# Autodesk Inventor assembly: Scrambler II
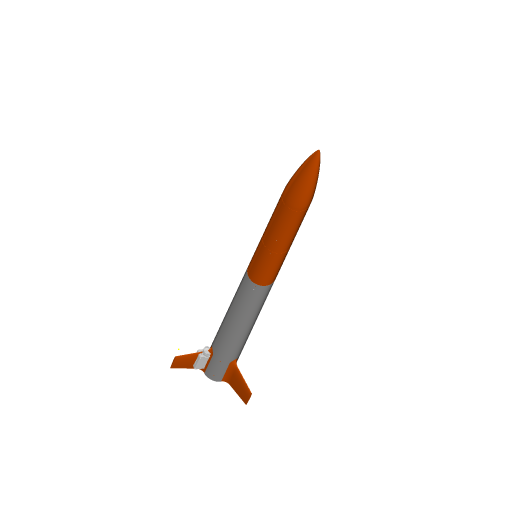
[picture p0: Inventor's stored thumbnail of the model, 512x512]
Saved by Autodesk Inventor 2024 (Build 280153000, 153)
## iProperties
Created: 2023-12-30
Part Number: Scrambler II
Document SubType Name: Assembly
Designer: Jamie
Mass: 631.455 g
Surface Area: 5625.65 cm^2
Volume: 391.502 cm^3
Density: 1.6129 g/cm^3
Author: Jamie
## Documents named in this file (7)
- C:\Users\Jamie\Documents\Uni\DARE\Scrambler-2-CAD\Autodesk\Scrambler II.iam
- C:\Users\Jamie\Documents\Uni\DARE\Scrambler-2-CAD\Autodesk\Structure.iam
- C:\Users\Jamie\Documents\Uni\DARE\Scrambler-2-CAD\Autodesk\Lower skin.ipt
- C:\Users\Jamie\Documents\Uni\DARE\Scrambler-2-CAD\Autodesk\Upper skin.ipt
- C:\Users\Jamie\Documents\Uni\DARE\Scrambler-2-CAD\Autodesk\Nosecone.ipt
- C:\Users\Jamie\Documents\Uni\DARE\Scrambler-2-CAD\Autodesk\SRM with Smoke Grain.iam
- C:\Users\Jamie\Documents\Uni\DARE\Scrambler-2-CAD\Autodesk\RunCam_HD2.ipt
## Components (6 placed, 6 different names)
1. Structure:1 [sub-assembly] — Mate:1, Mate:2, Mate:3, Mate:4, Mate:7, Mate:8
2. Lower skin:1 — Mate:1, Mate:2
3. Upper skin:1 — Mate:3, Mate:4, Mate:9, Mate:10, Mate:11
4. Nosecone:1 — Mate:9, Mate:10, Mate:11
5. SRM with Smoke Grain:1 [sub-assembly] — Mate:7, Mate:8
6. RunCam_HD2:1
## Relationships (9: Mate 9)
- Mate:1: Structure:1 ↔ Lower skin:1
- Mate:2: Structure:1 ↔ Lower skin:1
- Mate:3: Structure:1 ↔ Upper skin:1
- Mate:4: Structure:1 ↔ Upper skin:1
- Mate:7: Structure:1 ↔ SRM with Smoke Grain:1
- Mate:8: Structure:1 ↔ SRM with Smoke Grain:1
- Mate:9: Upper skin:1 ↔ Nosecone:1
- Mate:10: Upper skin:1 ↔ Nosecone:1
- Mate:11: Upper skin:1 ↔ Nosecone:1
